# Autodesk Inventor assembly: Gripper
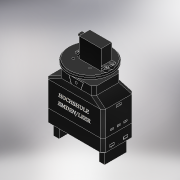
[picture p0: Inventor's stored thumbnail of the model, 180x180]
Saved by Autodesk Inventor 2022 (Build 260153000, 153)
## iProperties
Created: 2024-02-11
Part Number: Gripper
Document SubType Name: Assembly
Designer: alsaa
Author: alsaa
## Documents named in this file (11)
- C:\Users\alsaa\Desktop\Gripper\Gripper.iam
- C:\Users\alsaa\Desktop\Gripper\1.Holder_Part1.ipt
- C:\Users\alsaa\Desktop\Gripper\1.Holder_part2.ipt
- C:\Users\alsaa\Desktop\Gripper\2.Base.ipt
- C:\Users\alsaa\Desktop\Gripper\3.Case.ipt
- C:\Users\alsaa\Desktop\Gripper\4.Caver.ipt
- C:\Users\alsaa\Desktop\Gripper\5.Pinion.ipt
- C:\Users\alsaa\Desktop\Gripper\6.Rack.ipt
- C:\Users\alsaa\Desktop\Gripper\8.Rail.ipt
- C:\Users\alsaa\Desktop\Servo.ipt
- C:\Users\alsaa\Desktop\Gripper\9.Spacer.ipt
## Components (14 placed, 10 different names)
1. 1.Holder_Part1:1 — Fluchtend:1, Fluchtend:2, Passend:1, Passend:2, Passend:20, Passend:35
2. 1.Holder_part2:1 — Passend:2, Winkel:1, Winkel:2, Passend:4, Passend:7, Passend:20, Passend:36, Winkel:4
3. 2.Base:1 — Winkel:2, Passend:4, Passend:5, Passend:7, Passend:8
4. 3.Case:1 — Fluchtend:3, Passend:6, Passend:8, Passend:10
5. 4.Caver:1 — Passend:9, Fluchtend:4, Passend:10, Passend:11, Passend:12, Passend:15, Passend:16, Passend:18, Passend:19, Passend:21, Passend:22, Passend:25, Passend:26, Passend:27, Passend:28, Passend:29, Passend:30, Passend:31, Passend:32, Passend:33, Winkel:3, Passend:34
6. Stirnzahnrad1:1 — Passend:11, Passend:12, Fluchtend:14, Fluchtend:15, Passend:17
7. 6.Rack:1 — Fluchtend:14, Passend:15, Passend:19
8. 6.Rack:2 — Fluchtend:15, Passend:16, Passend:18, Passend:23, Passend:24
9. 8.Rail:1 — Passend:21, Passend:22, Passend:23, Passend:26
10. 8.Rail:2 — Passend:24, Passend:25
11. Servo:1 — Passend:33, Winkel:3, Passend:34
12. 9.Spacer:1 — Passend:27, Passend:28, Passend:29
13. 9.Spacer:2 — Passend:30, Passend:31, Passend:32
14. Servo:2 — Passend:35, Passend:36, Winkel:4
## Relationships (43: Mate 33, Flush 6, Angle 4)
- Fluchtend:1 [Flush]: 1.Holder_Part1:1
- Fluchtend:2 [Flush]: 1.Holder_Part1:1
- Passend:1 [Mate]: 1.Holder_Part1:1
- Passend:2 [Mate]: 1.Holder_Part1:1 ↔ 1.Holder_part2:1
- Winkel:1 [Angle] (180 deg): 1.Holder_part2:1
- Winkel:2 [Angle] (180 deg): 1.Holder_part2:1 ↔ 2.Base:1
- Passend:4 [Mate]: 1.Holder_part2:1 ↔ 2.Base:1
- Passend:5 [Mate]: 2.Base:1
- Fluchtend:3 [Flush]: 3.Case:1
- Passend:6 [Mate]: 3.Case:1
- Passend:7 [Mate]: 1.Holder_part2:1 ↔ 2.Base:1
- Passend:8 [Mate]: 2.Base:1 ↔ 3.Case:1
- Passend:9 [Mate]: 4.Caver:1
- Fluchtend:4 [Flush]: 4.Caver:1
- Passend:10 [Mate]: 3.Case:1 ↔ 4.Caver:1
- Passend:11 [Mate]: 4.Caver:1 ↔ Stirnzahnrad1:1
- Passend:12 [Mate]: 4.Caver:1 ↔ Stirnzahnrad1:1
- Fluchtend:14 [Flush]: Stirnzahnrad1:1 ↔ 6.Rack:1
- Fluchtend:15 [Flush]: Stirnzahnrad1:1 ↔ 6.Rack:2
- Passend:15 [Mate] (0.3 mm): 4.Caver:1 ↔ 6.Rack:1
- Passend:16 [Mate] (0.3 mm): 4.Caver:1 ↔ 6.Rack:2
- Passend:17 [Mate]: Stirnzahnrad1:1
- Passend:18 [Mate] (0.7 mm): 4.Caver:1 ↔ 6.Rack:2
- Passend:19 [Mate] (0.7 mm): 4.Caver:1 ↔ 6.Rack:1
- Passend:20 [Mate]: 1.Holder_Part1:1 ↔ 1.Holder_part2:1
- Passend:21 [Mate]: 4.Caver:1 ↔ 8.Rail:1
- Passend:22 [Mate]: 4.Caver:1 ↔ 8.Rail:1
- Passend:23 [Mate]: 6.Rack:2 ↔ 8.Rail:1
- Passend:24 [Mate]: 6.Rack:2 ↔ 8.Rail:2
- Passend:25 [Mate]: 4.Caver:1 ↔ 8.Rail:2
- Passend:26 [Mate]: 4.Caver:1 ↔ 8.Rail:1
- Passend:27 [Mate]: 4.Caver:1 ↔ 9.Spacer:1
- Passend:28 [Mate]: 4.Caver:1 ↔ 9.Spacer:1
- Passend:29 [Mate]: 4.Caver:1 ↔ 9.Spacer:1
- Passend:30 [Mate]: 4.Caver:1 ↔ 9.Spacer:2
- Passend:31 [Mate]: 4.Caver:1 ↔ 9.Spacer:2
- Passend:32 [Mate]: 4.Caver:1 ↔ 9.Spacer:2
- Passend:33 [Mate]: 4.Caver:1 ↔ Servo:1
- Winkel:3 [Angle] (0 deg): 4.Caver:1 ↔ Servo:1
- Passend:34 [Mate]: 4.Caver:1 ↔ Servo:1
- Passend:35 [Mate]: 1.Holder_Part1:1 ↔ Servo:2
- Passend:36 [Mate]: 1.Holder_part2:1 ↔ Servo:2
- Winkel:4 [Angle] (0 deg): 1.Holder_part2:1 ↔ Servo:2
## Named parameters: Abstand = 0 mm
